# Autodesk Inventor assembly: linear_cutting_endeffector
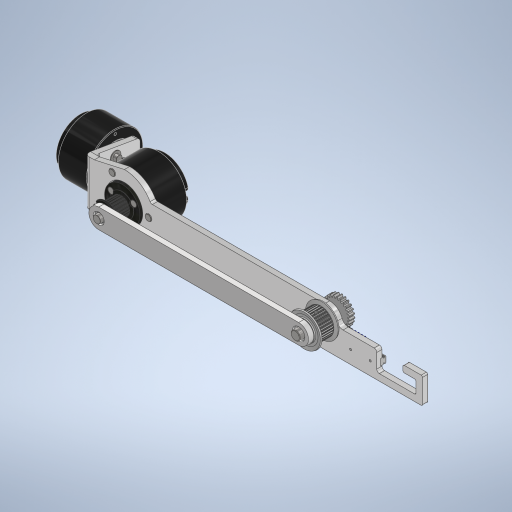
[picture p0: Inventor's stored thumbnail of the model, 512x512]
Saved by Autodesk Inventor 2024 (Build 280153000, 153)
## iProperties
Created: 2025-06-08
Part Number: linear_cutting_endeffector
Document SubType Name: Assembly
Designer: 1412z
Author: 1412z
## Documents named in this file (21)
- C:\Users\1412z\OneDrive\デスクトップ\rdclab\harvesting_robot\harvesting_endeffector\linear_cutting_endeffector\linear_cutting_endeffector.iam
- C:\Users\1412z\OneDrive\デスクトップ\rdclab\harvesting_robot\harvesting_endeffector\linear_cutting_endeffector\motor_holder\motor_holder.ipt
- C:\Users\1412z\OneDrive\デスクトップ\rdclab\harvesting_robot\harvesting_endeffector\linear_cutting_endeffector\misumi\SSE2B6L-100_Autodesk_Inventor_2023_20250607\AIS2023\SSE2B6-100_r.ipt
- C:\Users\1412z\OneDrive\デスクトップ\rdclab\harvesting_robot\harvesting_endeffector\linear_cutting_endeffector\misumi\SSE2B6L-100_Autodesk_Inventor_2023_20250607\AIS2023\SSEB6_b.ipt
- C:\Users\1412z\OneDrive\デスクトップ\rdclab\harvesting_robot\harvesting_endeffector\linear_cutting_endeffector\misumi\screw\NBK_SNZSM26\SNZS-M2-6.ipt
- C:\Users\1412z\OneDrive\デスクトップ\rdclab\harvesting_robot\harvesting_endeffector\linear_cutting_endeffector\misumi\LRGEAM0.8KA-80-K2-B50_Autodesk_Inventor_2024_20250607\LRGEAM0_8KA-80-K2-B50.ipt
- C:\Users\1412z\OneDrive\デスクトップ\rdclab\harvesting_robot\harvesting_endeffector\linear_cutting_endeffector\GIM3505-08\GIM3505-8_with-driver.ipt
- C:\Users\1412z\OneDrive\デスクトップ\rdclab\harvesting_robot\harvesting_endeffector\linear_cutting_endeffector\misumi\HTPA22S2M100-A-V4-Z6-J3_Autodesk_Inventor_2024_20250304\HTPA22S2M100-A-V4-Z6-J3_0_a-3.ipt
- C:\Users\1412z\OneDrive\デスクトップ\rdclab\harvesting_robot\harvesting_endeffector\linear_cutting_endeffector\misumi\screw\M2.5×4\M2.5×4.ipt
- C:\Users\1412z\OneDrive\デスクトップ\rdclab\harvesting_robot\harvesting_endeffector\linear_cutting_endeffector\misumi\washer\washer_M3.ipt
- C:\Users\1412z\OneDrive\デスクトップ\rdclab\harvesting_robot\harvesting_endeffector\linear_cutting_endeffector\misumi\C-FL675ZZ_Autodesk_Inventor_2024_20250608\C-FL675ZZ.ipt
- C:\Users\1412z\OneDrive\デスクトップ\rdclab\harvesting_robot\harvesting_endeffector\linear_cutting_endeffector\misumi\simring\simring_Φ5-Φ7.ipt
- C:\Users\1412z\OneDrive\デスクトップ\rdclab\harvesting_robot\harvesting_endeffector\linear_cutting_endeffector\misumi\HTPA32S2M100-A-P5_Autodesk_Inventor_2024_20250608\AIS2024\HTPA32S2M100-A-P5.iam
- C:\Users\1412z\OneDrive\デスクトップ\rdclab\harvesting_robot\harvesting_endeffector\linear_cutting_endeffector\motor_holder\motor_holder_top-2.ipt
- C:\Users\1412z\OneDrive\デスクトップ\rdclab\harvesting_robot\harvesting_endeffector\linear_cutting_endeffector\misumi\SFL674ZZ_Autodesk_Inventor_2024_20250304\SFL674ZZ.ipt
- C:\Users\1412z\OneDrive\デスクトップ\rdclab\harvesting_robot\harvesting_endeffector\linear_cutting_endeffector\misumi\screw\M3×8\M3×8.ipt
- C:\Users\1412z\OneDrive\デスクトップ\rdclab\harvesting_robot\harvesting_endeffector\linear_cutting_endeffector\misumi\shaft\shaft_15.05.ipt
- C:\Users\1412z\OneDrive\デスクトップ\rdclab\harvesting_robot\harvesting_endeffector\linear_cutting_endeffector\misumi\screw\M3×4\M3×4.ipt
- C:\Users\1412z\OneDrive\デスクトップ\rdclab\harvesting_robot\harvesting_endeffector\linear_cutting_endeffector\misumi\shaft\shaft_31.3mm_Φ5.ipt
- C:\Users\1412z\OneDrive\デスクトップ\rdclab\harvesting_robot\harvesting_endeffector\linear_cutting_endeffector\misumi\M0.8-24\Spur Gear (24 teeth).ipt
- C:\Users\1412z\OneDrive\デスクトップ\rdclab\harvesting_robot\harvesting_endeffector\linear_cutting_endeffector\misumi\screw\M4×5\M4×5.ipt
## Components (40 placed, 20 different names)
1. motor_holder:1 — 回転:1, 回転:2, 回転:15, 回転:16, 回転:17, 回転:18, 回転:21, 回転:22, 回転:23, 回転:30, 回転:31, 回転:32, 回転:33
2. SSE2B6-100_r:1 — 回転:1, 回転:2, 回転:3, 回転:4, 回転:5, リジッド:1, 回転:6, 回転:7, 回転:8, 円柱状:1, 円柱状:2
3. SNZS-M2-6:1 — 回転:3
4. SNZS-M2-6:2 — 回転:4
5. SNZS-M2-6:3 — リジッド:1
6. SNZS-M2-6:4 — 回転:8
7. SNZS-M2-6:5 — 回転:7
8. SNZS-M2-6:6 — 回転:6
9. SNZS-M2-6:7 — 回転:5
10. SSEB6_b:1 — 円柱状:1, 回転:10
11. SSEB6_b:2 — 円柱状:2, 回転:9
12. LRGEAM0_8KA-80-K2-B50:1 — 回転:9, 回転:10
13. GIM3505-8_with-driver:1 — 回転:15, 回転:16, 回転:19, 回転:20
14. GIM3505-8_with-driver:2 — 回転:17, 回転:18
15. HTPA22S2M100-A-V4-Z6-J3_0_a-3:1 — 回転:19, 回転:20, 回転:27, 回転:28, 回転:29, 回転:37, 回転:40
16. M2.5×4:1 — 回転:27
17. M2.5×4:2 — 回転:28
18. M2.5×4:3 — 回転:29
19. M2.5×4:4 — 回転:24
20. M2.5×4:5 — 回転:25
21. M2.5×4:6 — 回転:26
22. washer_M3:1 — 回転:21, 回転:24
23. washer_M3:2 — 回転:23, 回転:26
24. washer_M3:3 — 回転:22, 回転:25
25. M2.5×4:7 — 回転:31
26. M2.5×4:8 — 回転:30
27. M2.5×4:9 — 回転:32
28. C-FL675ZZ:2 — 回転:33, 回転:34
29. simring_Φ5-Φ7:1 — 回転:34, 回転:35
30. HTPA32S2M100-A-P5:1 [sub-assembly] — 回転:35, 回転:36
31. motor_holder_top-2:1 — 回転:36, 回転:37, 回転:38, 回転:39
32. C-FL675ZZ:3 — 回転:38, 回転:43
33. SFL674ZZ:1 — 回転:39, 回転:41
34. M3×8:1 — リジッド:2
35. washer_M3:4 — 回転:40, リジッド:2
36. shaft_15.05:1 — 回転:41, 回転:42
37. M3×4:1 — 回転:42
38. shaft_31.3mm_Φ5:1 — 回転:43, 回転:44, 回転:45
39. Spur Gear (24 teeth):1 — 回転:44
40. M4×5:1 — 回転:45
## Relationships (45: RevoluteJoint 41, WeldJoint 2, CylindricalJoint 2)
- 回転:1 [RevoluteJoint]: motor_holder:1 ↔ SSE2B6-100_r:1
- 回転:2 [RevoluteJoint]: motor_holder:1 ↔ SSE2B6-100_r:1
- 回転:3 [RevoluteJoint]: SSE2B6-100_r:1 ↔ SNZS-M2-6:1
- 回転:4 [RevoluteJoint]: SSE2B6-100_r:1 ↔ SNZS-M2-6:2
- 回転:5 [RevoluteJoint]: SSE2B6-100_r:1 ↔ SNZS-M2-6:7
- リジッド:1 [WeldJoint]: SSE2B6-100_r:1 ↔ SNZS-M2-6:3
- 回転:6 [RevoluteJoint]: SSE2B6-100_r:1 ↔ SNZS-M2-6:6
- 回転:7 [RevoluteJoint]: SSE2B6-100_r:1 ↔ SNZS-M2-6:5
- 回転:8 [RevoluteJoint]: SSE2B6-100_r:1 ↔ SNZS-M2-6:4
- 円柱状:1 [CylindricalJoint]: SSE2B6-100_r:1 ↔ SSEB6_b:1
- 円柱状:2 [CylindricalJoint]: SSE2B6-100_r:1 ↔ SSEB6_b:2
- 回転:9 [RevoluteJoint]: SSEB6_b:2 ↔ LRGEAM0_8KA-80-K2-B50:1
- 回転:10 [RevoluteJoint]: SSEB6_b:1 ↔ LRGEAM0_8KA-80-K2-B50:1
- 回転:15 [RevoluteJoint]: motor_holder:1 ↔ GIM3505-8_with-driver:1
- 回転:16 [RevoluteJoint]: motor_holder:1 ↔ GIM3505-8_with-driver:1
- 回転:17 [RevoluteJoint]: motor_holder:1 ↔ GIM3505-8_with-driver:2
- 回転:18 [RevoluteJoint]: motor_holder:1 ↔ GIM3505-8_with-driver:2
- 回転:19 [RevoluteJoint]: GIM3505-8_with-driver:1 ↔ HTPA22S2M100-A-V4-Z6-J3_0_a-3:1
- 回転:20 [RevoluteJoint]: GIM3505-8_with-driver:1 ↔ HTPA22S2M100-A-V4-Z6-J3_0_a-3:1
- 回転:21 [RevoluteJoint]: motor_holder:1 ↔ washer_M3:1
- 回転:22 [RevoluteJoint]: motor_holder:1 ↔ washer_M3:3
- 回転:23 [RevoluteJoint]: motor_holder:1 ↔ washer_M3:2
- 回転:24 [RevoluteJoint]: M2.5×4:4 ↔ washer_M3:1
- 回転:25 [RevoluteJoint]: M2.5×4:5 ↔ washer_M3:3
- 回転:26 [RevoluteJoint]: M2.5×4:6 ↔ washer_M3:2
- 回転:27 [RevoluteJoint]: HTPA22S2M100-A-V4-Z6-J3_0_a-3:1 ↔ M2.5×4:1
- 回転:28 [RevoluteJoint]: HTPA22S2M100-A-V4-Z6-J3_0_a-3:1 ↔ M2.5×4:2
- 回転:29 [RevoluteJoint]: HTPA22S2M100-A-V4-Z6-J3_0_a-3:1 ↔ M2.5×4:3
- 回転:30 [RevoluteJoint]: motor_holder:1 ↔ M2.5×4:8
- 回転:31 [RevoluteJoint]: motor_holder:1 ↔ M2.5×4:7
- 回転:32 [RevoluteJoint]: motor_holder:1 ↔ M2.5×4:9
- 回転:33 [RevoluteJoint]: motor_holder:1 ↔ C-FL675ZZ:2
- 回転:34 [RevoluteJoint]: C-FL675ZZ:2 ↔ simring_Φ5-Φ7:1
- 回転:35 [RevoluteJoint]: simring_Φ5-Φ7:1 ↔ HTPA32S2M100-A-P5:1
- 回転:36 [RevoluteJoint]: HTPA32S2M100-A-P5:1 ↔ motor_holder_top-2:1
- 回転:37 [RevoluteJoint]: HTPA22S2M100-A-V4-Z6-J3_0_a-3:1 ↔ motor_holder_top-2:1
- 回転:38 [RevoluteJoint]: motor_holder_top-2:1 ↔ C-FL675ZZ:3
- 回転:39 [RevoluteJoint]: motor_holder_top-2:1 ↔ SFL674ZZ:1
- 回転:40 [RevoluteJoint]: HTPA22S2M100-A-V4-Z6-J3_0_a-3:1 ↔ washer_M3:4
- 回転:41 [RevoluteJoint]: SFL674ZZ:1 ↔ shaft_15.05:1
- リジッド:2 [WeldJoint]: M3×8:1 ↔ washer_M3:4
- 回転:42 [RevoluteJoint]: shaft_15.05:1 ↔ M3×4:1
- 回転:43 [RevoluteJoint]: C-FL675ZZ:3 ↔ shaft_31.3mm_Φ5:1
- 回転:44 [RevoluteJoint]: shaft_31.3mm_Φ5:1 ↔ Spur Gear (24 teeth):1
- 回転:45 [RevoluteJoint]: shaft_31.3mm_Φ5:1 ↔ M4×5:1
